# Autodesk Inventor assembly: Final AssemblyV5
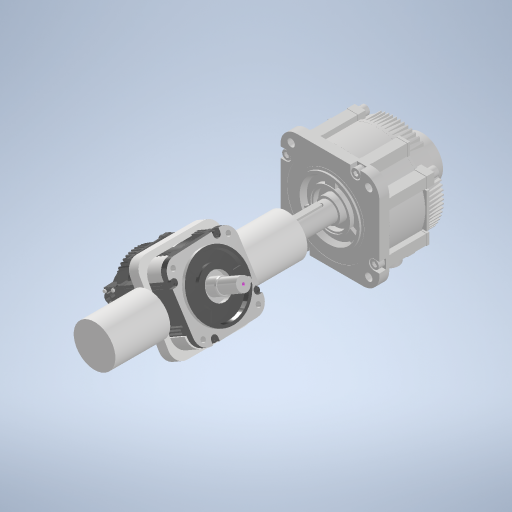
[picture p0: Inventor's stored thumbnail of the model, 512x512]
Saved by Autodesk Inventor 2024 (Build 280153000, 153)
## iProperties
Created: 2024-02-08
Part Number: Final AssemblyV5
Document SubType Name: Assembly
Designer: yusuf
Author: yusuf
## Documents named in this file (4)
- C:\Users\yusuf\Documents\DodgeBot\CAD_FILES\Final AssemblyV5.iam
- C:\Users\yusuf\Documents\DodgeBot\CAD_FILES\YASKAWA_USA_SGM7G30A6A61\AIS2024\SGM7G-30A6A61.iam
- C:\Users\yusuf\Documents\DodgeBot\CAD_FILES\FrontPlateV2.ipt
- C:\Users\yusuf\Documents\DodgeBot\CAD_FILES\SGM7G_20AxA61\SGM7G-20xxA61\ProE\SGM7G-20__a61_ProE\ProE\sgm7g_20__a61\sgm7g_20__a61.iam
## Components (3 placed, 3 different names)
1. SGM7G-30A6A61:1 [sub-assembly] — Rotational:2
2. FrontPlateV2:1 — Rotational:2, Rigid:1
3. sgm7g_20__a61:1 [sub-assembly] — Rigid:1
## Relationships (2: RevoluteJoint 1, WeldJoint 1)
- Rotational:2 [RevoluteJoint]: SGM7G-30A6A61:1 ↔ FrontPlateV2:1
- Rigid:1 [WeldJoint]: FrontPlateV2:1 ↔ sgm7g_20__a61:1
